# Autodesk Inventor assembly: pixel
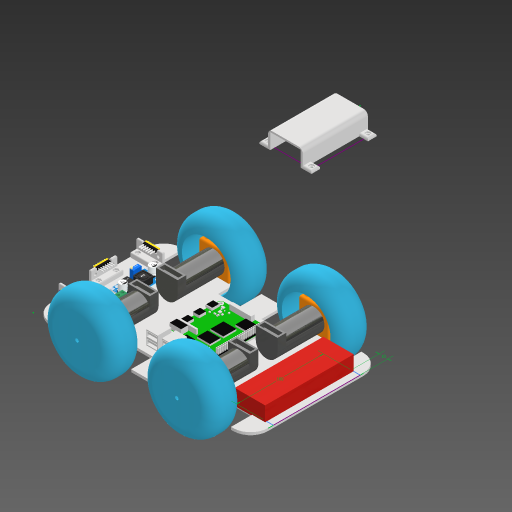
[picture p0: Inventor's stored thumbnail of the model, 512x512]
Saved by Autodesk Inventor 2023 (Build 270158000, 158)
## iProperties
Created: 2025-08-08
Part Number: pixel
Document SubType Name: Assembly
Designer: daa
Author: daa
## Documents named in this file (12)
- C:\Users\daa\Documents\DASH_V2\omni_platforma\pixel.iam
- C:\Users\daa\Documents\RTC\niz.ipt
- C:\Users\daa\Documents\RTC\motor.ipt
- C:\Users\daa\Documents\RTC\motor25.ipt
- C:\Users\daa\Documents\RTC\wheel_85.ipt
- C:\Users\daa\Documents\RTC\raspberrypi.ipt
- C:\Users\daa\Documents\RTC\VL53L0.ipt
- C:\Users\daa\Documents\RTC\vl53l0_mount.ipt
- C:\Users\daa\Documents\RTC\L9110S Motor Driver.ipt
- C:\Users\daa\Documents\RTC\LM256.iam
- C:\Users\daa\Documents\RTC\akb.ipt
- C:\Users\daa\Documents\RTC\akb_mount.ipt
## Components (24 placed, 11 different names)
1. niz:1 — Совмещение:1, Совмещение:2, Совмещение:3, Совмещение:4, Совмещение:5, Совмещение:6, Совмещение:7, Совмещение:8, Совмещение:9, Совмещение:10, Совмещение:11, Совмещение:12, Совмещение:16, Совмещение:17
2. motor:1 — Совмещение:1, Совмещение:2, С поворотом:2
3. motor25:1 — С поворотом:2, С поворотом:8
4. motor:2 — Совмещение:6, С поворотом:4
5. motor25:2 — С поворотом:1, С поворотом:7
6. motor:3 — Совмещение:5, С поворотом:3
7. motor25:3 — С поворотом:3, С поворотом:5
8. motor:4 — Совмещение:3, Совмещение:4, С поворотом:1
9. motor25:4 — С поворотом:4, С поворотом:6
10. wheel_85:1 — С поворотом:8
11. wheel_85:2 — С поворотом:6
12. wheel_85:3 — С поворотом:5
13. wheel_85:4 — С поворотом:7
14. raspberrypi:1 — Совмещение:7
15. VL53L0:1 — Совмещение:13
16. vl53l0_mount:1 — Совмещение:9, Совмещение:10, Совмещение:15
17. VL53L0:2 — Совмещение:14
18. vl53l0_mount:2 — Совмещение:8, Совмещение:14
19. VL53L0:3 — Совмещение:15
20. vl53l0_mount:3 — Совмещение:11, Совмещение:12, Совмещение:13
21. L9110S Motor Driver:1 — Совмещение:17
22. LM256:1 [sub-assembly] — Совмещение:16
23. akb:1
24. akb_mount:1
## Relationships (25: Mate 17, RevoluteJoint 8)
- Совмещение:1 [Mate]: niz:1 ↔ motor:1
- Совмещение:2 [Mate]: niz:1 ↔ motor:1
- Совмещение:3 [Mate]: niz:1 ↔ motor:4
- Совмещение:4 [Mate]: niz:1 ↔ motor:4
- Совмещение:5 [Mate]: niz:1 ↔ motor:3
- Совмещение:6 [Mate]: niz:1 ↔ motor:2
- С поворотом:1 [RevoluteJoint] (-7 mm): motor25:2 ↔ motor:4
- С поворотом:2 [RevoluteJoint] (-7 mm): motor:1 ↔ motor25:1
- С поворотом:3 [RevoluteJoint] (-7 mm): motor:3 ↔ motor25:3
- С поворотом:4 [RevoluteJoint] (-7 mm): motor:2 ↔ motor25:4
- С поворотом:5 [RevoluteJoint] (-5.5 mm): motor25:3 ↔ wheel_85:3
- С поворотом:6 [RevoluteJoint] (-5.5 mm): motor25:4 ↔ wheel_85:2
- С поворотом:7 [RevoluteJoint] (-5.5 mm): motor25:2 ↔ wheel_85:4
- С поворотом:8 [RevoluteJoint] (-5.5 mm): motor25:1 ↔ wheel_85:1
- Совмещение:7 [Mate]: niz:1 ↔ raspberrypi:1
- Совмещение:8 [Mate]: niz:1 ↔ vl53l0_mount:2
- Совмещение:9 [Mate]: niz:1 ↔ vl53l0_mount:1
- Совмещение:10 [Mate]: niz:1 ↔ vl53l0_mount:1
- Совмещение:11 [Mate]: niz:1 ↔ vl53l0_mount:3
- Совмещение:12 [Mate]: niz:1 ↔ vl53l0_mount:3
- Совмещение:13 [Mate]: VL53L0:1 ↔ vl53l0_mount:3
- Совмещение:14 [Mate]: VL53L0:2 ↔ vl53l0_mount:2
- Совмещение:15 [Mate]: vl53l0_mount:1 ↔ VL53L0:3
- Совмещение:16 [Mate]: niz:1 ↔ LM256:1
- Совмещение:17 [Mate]: niz:1 ↔ L9110S Motor Driver:1
